# Autodesk Inventor assembly: サス
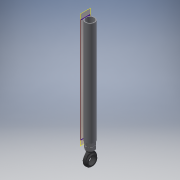
[picture p0: Inventor's stored thumbnail of the model, 180x180]
Saved by Autodesk Inventor 2018 (Build 220112000, 112)
## iProperties
Created: 2017-09-07
Part Number: サス
Material: 一般
Document SubType Name: Assembly
Designer: Kosei
Author: Kosei
## Documents named in this file (4)
- C:\Users\mura5\Documents\RBBR\cart\Rod1.iam
- C:\Users\mura5\Documents\RBBR\cart\Pipe1.ipt
- C:\Users\mura5\Documents\RBBR\cart\hn1_14.ipt
- C:\Users\mura5\Documents\RBBR\cart\iko_POS_14EC\AIS2016\POS 14ECBody.ipt
## Components (4 placed, 3 different names)
1. Pipe1:1 — リジッド:2
2. hn1_14:2 — リジッド:2, 回転:1
3. POS 14ECBody:1
4. hn1_14:3 — 回転:1
## Relationships (3: WeldJoint 2, RevoluteJoint 1)
- リジッド:2 [WeldJoint]: Pipe1:1 ↔ hn1_14:2
- [WeldJoint] (15 mm): hn1_14:2 ↔ POS 14ECBody:1
- 回転:1 [RevoluteJoint]: hn1_14:2 ↔ hn1_14:3
